# Autodesk Inventor assembly: MainAssemblie
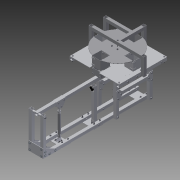
[picture p0: Inventor's stored thumbnail of the model, 180x180]
Saved by Autodesk Inventor 2013 (Build 170138000, 138)
## iProperties
Created: 2013-07-15
Part Number: MainAssemblie
Document SubType Name: Assembly
Designer: root
Mass: 9552.06 g
Surface Area: 27786.8 cm^2
Volume: 3156.7 cm^3
Density: 3.02596 g/cm^3
Author: root
## Documents named in this file (15)
- I:\FRC_Projects\Cad\Inventor_Projects\Shooter_No_Welding\MainAssemblie.iam
- I:\FRC_Projects\Cad\Inventor_Projects\Shooter_No_Welding\Base\BaseAssemblies.iam
- I:\FRC_Projects\Cad\Inventor_Projects\Shooter_No_Welding\Thrower\ThrowerAssemblie.iam
- I:\FRC_Projects\Cad\Inventor_Projects\Shooter_No_Welding\Hopper\HopperAssembly.iam
- I:\FRC_Projects\Cad\Inventor_Projects\Shooter_No_Welding\Thrower\cylinder\045_DP_D_167__F_D_166_3__2_14b.iam
- I:\FRC_Projects\Cad\Inventor_Projects\Shooter_No_Welding\Thrower\cylinder\5.ipt
- I:\FRC_Projects\Cad\Inventor_Projects\Shooter_No_Welding\Thrower\cylinder\6.ipt
- I:\FRC_Projects\Cad\Inventor_Projects\Shooter_No_Welding\contentCenter\en-US\ANSI B18.2.2(09)\ANSI B18.2.2 - 1_4 - 20(2).ipt
- I:\FRC_Projects\Cad\Inventor_Projects\Shooter_No_Welding\contentCenter\en-US\ANSI ASME B18.2.1(2)\ANSI_ASME B18.2.1 - 1_4-20 UNC - 2.25(2).ipt
- I:\FRC_Projects\Cad\Inventor_Projects\Shooter_No_Welding\contentCenter\en-US\ANSI ASME B18.2.1(2)\ANSI_ASME B18.2.1 - 1_4-20 UNC - 0.75(2).ipt
- I:\FRC_Projects\Cad\Inventor_Projects\Shooter_No_Welding\contentCenter\en-US\ASTM F436(1)\ASTM F436 - 1_4(1).ipt
- I:\FRC_Projects\Cad\Inventor_Projects\Shooter_No_Welding\Thrower\cylinder\4.ipt
- I:\FRC_Projects\Cad\Inventor_Projects\Shooter_No_Welding\contentCenter\en-US\ANSI ASME B18.2.1(2)\ANSI_ASME B18.2.1 - 1_4-20 UNC - 1.75(2).ipt
- I:\FRC_Projects\Cad\Inventor_Projects\Shooter_No_Welding\Thrower\ModdedSEN_Microswitch_V7-2B17D8-048.ipt
- I:\FRC_Projects\Cad\Inventor_Projects\Shooter_No_Welding\contentCenter\en-US\ANSI ASME B18.2.1(2)\ANSI_ASME B18.2.1 - 1_4-20 UNC - 1.5(2).ipt
## Components (43 placed, 14 different names)
1. BaseAssemblies:1 [sub-assembly] — Mate:1, Mate:2, Mate:3, Mate:4, Flush:1, Mate:7, Mate:8, Mate:9, Mate:13, Mate:18, Mate:19, Mate:23, Mate:25, Mate:27, Mate:29, Mate:30, Mate:31, Mate:32, Mate:33, Mate:34, Mate:35, Mate:36, Mate:37, Mate:38, Mate:68, Angle:1, Mate:69, Mate:70, Mate:71, Mate:72, Mate:73, Mate:74, Mate:75, Mate:76, Mate:77, Mate:82, Mate:83, Mate:84, Mate:85
2. ThrowerAssemblie:1 [sub-assembly] — Mate:1, Mate:2, Mate:11, Mate:12
3. HopperAssembly:1 [sub-assembly] — Mate:3, Mate:4, Flush:1, Mate:13, Mate:14, Mate:15, Mate:16, Mate:17, Mate:20, Mate:21, Mate:56, Mate:57, Mate:58, Mate:59, Mate:60, Mate:61, Mate:86, Mate:87, Mate:88
4. 5:1 — Mate:5, Mate:6, Flush:3, Mate:7, Mate:40, Mate:42
5. 6:1 — Mate:5, Mate:6, Flush:3, Mate:8, Mate:9, Mate:10, Mate:44, Mate:52, Mate:54, Mate:55, Flush:4
6. 045_DP_D_167__F_D_166_3__2_14b:1 [sub-assembly] — Mate:10, Mate:11, Mate:12
7. Hex Nut - Inch 1/4 - 20:1 — Mate:28, Mate:29
8. Hex Nut - Inch 1/4 - 20:2 — Mate:26, Mate:27
9. Hex Nut - Inch 1/4 - 20:3 — Mate:24, Mate:25
10. Hex Nut - Inch 1/4 - 20:4 — Mate:22, Mate:23
11. Hex Bolt - Inch 1/4-20 UNC - 2.25:1 — Mate:15, Mate:17, Mate:28
12. Hex Bolt - Inch 1/4-20 UNC - 2.25:2 — Mate:18, Mate:21, Mate:24
13. Hex Bolt - Inch 1/4-20 UNC - 2.25:3 — Mate:14, Mate:16, Mate:22
14. Hex Bolt - Inch 1/4-20 UNC - 2.25:4 — Mate:19, Mate:20, Mate:26
15. Hex Bolt - Inch 1/4-20 UNC - 0.75:1 — Mate:31, Mate:34, Mate:43, Mate:49
16. Hex Bolt - Inch 1/4-20 UNC - 0.75:2 — Mate:32, Mate:35, Mate:51, Mate:53
17. Hex Bolt - Inch 1/4-20 UNC - 0.75:3 — Mate:36
18. Hex Bolt - Inch 1/4-20 UNC - 0.75:4 — Mate:30, Mate:33, Mate:41, Mate:47
19. Hex Bolt - Inch 1/4-20 UNC - 0.75:5 — Mate:37, Mate:38, Mate:39, Mate:45
20. Hex Nut - Inch 1/4 - 20:5 — Mate:53, Mate:54
21. Hex Nut - Inch 1/4 - 20:6 — Mate:49, Mate:50
22. Hex Nut - Inch 1/4 - 20:7 — Mate:47, Mate:48
23. Hex Nut - Inch 1/4 - 20:8 — Mate:45, Mate:46
24. Circular Washer (Inch) 1/4:1 — Mate:39, Mate:40, Mate:46
25. Circular Washer (Inch) 1/4:2 — Mate:51, Mate:52
26. Circular Washer (Inch) 1/4:3 — Mate:43, Mate:44, Mate:50
27. Circular Washer (Inch) 1/4:4 — Mate:41, Mate:42, Mate:48
28. 4:1 — Mate:55, Flush:4
29. Hex Bolt - Inch 1/4-20 UNC - 1.75:1 — Mate:58, Mate:59, Mate:64
30. Hex Bolt - Inch 1/4-20 UNC - 1.75:2 — Mate:60, Mate:61, Mate:63
31. Hex Bolt - Inch 1/4-20 UNC - 1.75:3 — Mate:56, Mate:57, Mate:62
32. Hex Nut - Inch 1/4 - 20:9 — Mate:64, Mate:88
33. Hex Nut - Inch 1/4 - 20:10 — Mate:63, Mate:87
34. Hex Nut - Inch 1/4 - 20:11 — Mate:62, Mate:86
35. ModdedSEN_Microswitch_V7-2B17D8-048:1 — Mate:68, Angle:1, Mate:69
36. Hex Bolt - Inch 1/4-20 UNC - 1.5:1 — Mate:73, Mate:75, Mate:79
37. Hex Bolt - Inch 1/4-20 UNC - 1.5:2 — Mate:72, Mate:74, Mate:78
38. Hex Bolt - Inch 1/4-20 UNC - 1.5:3 — Mate:70, Mate:76, Mate:81
39. Hex Bolt - Inch 1/4-20 UNC - 1.5:4 — Mate:71, Mate:77, Mate:80
40. Hex Nut - Inch 1/4 - 20:12 — Mate:81, Mate:84
41. Hex Nut - Inch 1/4 - 20:13 — Mate:79, Mate:83
42. Hex Nut - Inch 1/4 - 20:14 — Mate:80, Mate:85
43. Hex Nut - Inch 1/4 - 20:15 — Mate:78, Mate:82
## Relationships (89: Mate 85, Flush 3, Angle 1)
- Mate:1: BaseAssemblies:1 ↔ ThrowerAssemblie:1
- Mate:2: BaseAssemblies:1 ↔ ThrowerAssemblie:1
- Mate:3: BaseAssemblies:1 ↔ HopperAssembly:1
- Mate:4: BaseAssemblies:1 ↔ HopperAssembly:1
- Flush:1: BaseAssemblies:1 ↔ HopperAssembly:1
- Mate:5 (9.525 mm): 5:1 ↔ 6:1
- Mate:6: 5:1 ↔ 6:1
- Flush:3: 5:1 ↔ 6:1
- Mate:7: BaseAssemblies:1 ↔ 5:1
- Mate:8 (184.15 mm): BaseAssemblies:1 ↔ 6:1
- Mate:9 (42.8625 mm): BaseAssemblies:1 ↔ 6:1
- Mate:10: 6:1 ↔ 045_DP_D_167__F_D_166_3__2_14b:1
- Mate:11: ThrowerAssemblie:1 ↔ 045_DP_D_167__F_D_166_3__2_14b:1
- Mate:12: ThrowerAssemblie:1 ↔ 045_DP_D_167__F_D_166_3__2_14b:1
- Mate:13: BaseAssemblies:1 ↔ HopperAssembly:1
- Mate:14: HopperAssembly:1 ↔ Hex Bolt - Inch 1/4-20 UNC - 2.25:3
- Mate:15: HopperAssembly:1 ↔ Hex Bolt - Inch 1/4-20 UNC - 2.25:1
- Mate:16: HopperAssembly:1 ↔ Hex Bolt - Inch 1/4-20 UNC - 2.25:3
- Mate:17: HopperAssembly:1 ↔ Hex Bolt - Inch 1/4-20 UNC - 2.25:1
- Mate:18: BaseAssemblies:1 ↔ Hex Bolt - Inch 1/4-20 UNC - 2.25:2
- Mate:19: BaseAssemblies:1 ↔ Hex Bolt - Inch 1/4-20 UNC - 2.25:4
- Mate:20: HopperAssembly:1 ↔ Hex Bolt - Inch 1/4-20 UNC - 2.25:4
- Mate:21: HopperAssembly:1 ↔ Hex Bolt - Inch 1/4-20 UNC - 2.25:2
- Mate:22: Hex Nut - Inch 1/4 - 20:4 ↔ Hex Bolt - Inch 1/4-20 UNC - 2.25:3
- Mate:23: BaseAssemblies:1 ↔ Hex Nut - Inch 1/4 - 20:4
- Mate:24: Hex Nut - Inch 1/4 - 20:3 ↔ Hex Bolt - Inch 1/4-20 UNC - 2.25:2
- Mate:25: BaseAssemblies:1 ↔ Hex Nut - Inch 1/4 - 20:3
- Mate:26: Hex Nut - Inch 1/4 - 20:2 ↔ Hex Bolt - Inch 1/4-20 UNC - 2.25:4
- Mate:27: BaseAssemblies:1 ↔ Hex Nut - Inch 1/4 - 20:2
- Mate:28: Hex Nut - Inch 1/4 - 20:1 ↔ Hex Bolt - Inch 1/4-20 UNC - 2.25:1
- Mate:29: BaseAssemblies:1 ↔ Hex Nut - Inch 1/4 - 20:1
- Mate:30: BaseAssemblies:1 ↔ Hex Bolt - Inch 1/4-20 UNC - 0.75:4
- Mate:31: BaseAssemblies:1 ↔ Hex Bolt - Inch 1/4-20 UNC - 0.75:1
- Mate:32: BaseAssemblies:1 ↔ Hex Bolt - Inch 1/4-20 UNC - 0.75:2
- Mate:33: BaseAssemblies:1 ↔ Hex Bolt - Inch 1/4-20 UNC - 0.75:4
- Mate:34: BaseAssemblies:1 ↔ Hex Bolt - Inch 1/4-20 UNC - 0.75:1
- Mate:35: BaseAssemblies:1 ↔ Hex Bolt - Inch 1/4-20 UNC - 0.75:2
- Mate:36: BaseAssemblies:1 ↔ Hex Bolt - Inch 1/4-20 UNC - 0.75:3
- Mate:37: BaseAssemblies:1 ↔ Hex Bolt - Inch 1/4-20 UNC - 0.75:5
- Mate:38: BaseAssemblies:1 ↔ Hex Bolt - Inch 1/4-20 UNC - 0.75:5
- Mate:39: Hex Bolt - Inch 1/4-20 UNC - 0.75:5 ↔ Circular Washer (Inch) 1/4:1
- Mate:40: 5:1 ↔ Circular Washer (Inch) 1/4:1
- Mate:41: Hex Bolt - Inch 1/4-20 UNC - 0.75:4 ↔ Circular Washer (Inch) 1/4:4
- Mate:42: 5:1 ↔ Circular Washer (Inch) 1/4:4
- Mate:43: Hex Bolt - Inch 1/4-20 UNC - 0.75:1 ↔ Circular Washer (Inch) 1/4:3
- Mate:44: 6:1 ↔ Circular Washer (Inch) 1/4:3
- Mate:45: Hex Bolt - Inch 1/4-20 UNC - 0.75:5 ↔ Hex Nut - Inch 1/4 - 20:8
- Mate:46: Hex Nut - Inch 1/4 - 20:8 ↔ Circular Washer (Inch) 1/4:1
- Mate:47: Hex Bolt - Inch 1/4-20 UNC - 0.75:4 ↔ Hex Nut - Inch 1/4 - 20:7
- Mate:48: Hex Nut - Inch 1/4 - 20:7 ↔ Circular Washer (Inch) 1/4:4
- Mate:49: Hex Bolt - Inch 1/4-20 UNC - 0.75:1 ↔ Hex Nut - Inch 1/4 - 20:6
- Mate:50: Hex Nut - Inch 1/4 - 20:6 ↔ Circular Washer (Inch) 1/4:3
- Mate:51: Hex Bolt - Inch 1/4-20 UNC - 0.75:2 ↔ Circular Washer (Inch) 1/4:2
- Mate:52: 6:1 ↔ Circular Washer (Inch) 1/4:2
- Mate:53: Hex Bolt - Inch 1/4-20 UNC - 0.75:2 ↔ Hex Nut - Inch 1/4 - 20:5
- Mate:54: 6:1 ↔ Hex Nut - Inch 1/4 - 20:5
- Mate:55: 6:1 ↔ 4:1
- Flush:4: 6:1 ↔ 4:1
- Mate:56: HopperAssembly:1 ↔ Hex Bolt - Inch 1/4-20 UNC - 1.75:3
- Mate:57: HopperAssembly:1 ↔ Hex Bolt - Inch 1/4-20 UNC - 1.75:3
- Mate:58: HopperAssembly:1 ↔ Hex Bolt - Inch 1/4-20 UNC - 1.75:1
- Mate:59: HopperAssembly:1 ↔ Hex Bolt - Inch 1/4-20 UNC - 1.75:1
- Mate:60: HopperAssembly:1 ↔ Hex Bolt - Inch 1/4-20 UNC - 1.75:2
- Mate:61: HopperAssembly:1 ↔ Hex Bolt - Inch 1/4-20 UNC - 1.75:2
- Mate:62: Hex Bolt - Inch 1/4-20 UNC - 1.75:3 ↔ Hex Nut - Inch 1/4 - 20:11
- Mate:63: Hex Bolt - Inch 1/4-20 UNC - 1.75:2 ↔ Hex Nut - Inch 1/4 - 20:10
- Mate:64: Hex Bolt - Inch 1/4-20 UNC - 1.75:1 ↔ Hex Nut - Inch 1/4 - 20:9
- Mate:68: BaseAssemblies:1 ↔ ModdedSEN_Microswitch_V7-2B17D8-048:1
- Angle:1 (-45 deg): BaseAssemblies:1 ↔ ModdedSEN_Microswitch_V7-2B17D8-048:1
- Mate:69: BaseAssemblies:1 ↔ ModdedSEN_Microswitch_V7-2B17D8-048:1
- Mate:70: BaseAssemblies:1 ↔ Hex Bolt - Inch 1/4-20 UNC - 1.5:3
- Mate:71: BaseAssemblies:1 ↔ Hex Bolt - Inch 1/4-20 UNC - 1.5:4
- Mate:72: BaseAssemblies:1 ↔ Hex Bolt - Inch 1/4-20 UNC - 1.5:2
- Mate:73: BaseAssemblies:1 ↔ Hex Bolt - Inch 1/4-20 UNC - 1.5:1
- Mate:74: BaseAssemblies:1 ↔ Hex Bolt - Inch 1/4-20 UNC - 1.5:2
- Mate:75: BaseAssemblies:1 ↔ Hex Bolt - Inch 1/4-20 UNC - 1.5:1
- Mate:76: BaseAssemblies:1 ↔ Hex Bolt - Inch 1/4-20 UNC - 1.5:3
- Mate:77: BaseAssemblies:1 ↔ Hex Bolt - Inch 1/4-20 UNC - 1.5:4
- Mate:78: Hex Bolt - Inch 1/4-20 UNC - 1.5:2 ↔ Hex Nut - Inch 1/4 - 20:15
- Mate:79: Hex Bolt - Inch 1/4-20 UNC - 1.5:1 ↔ Hex Nut - Inch 1/4 - 20:13
- Mate:80: Hex Bolt - Inch 1/4-20 UNC - 1.5:4 ↔ Hex Nut - Inch 1/4 - 20:14
- Mate:81: Hex Bolt - Inch 1/4-20 UNC - 1.5:3 ↔ Hex Nut - Inch 1/4 - 20:12
- Mate:82: BaseAssemblies:1 ↔ Hex Nut - Inch 1/4 - 20:15
- Mate:83: BaseAssemblies:1 ↔ Hex Nut - Inch 1/4 - 20:13
- Mate:84: BaseAssemblies:1 ↔ Hex Nut - Inch 1/4 - 20:12
- Mate:85: BaseAssemblies:1 ↔ Hex Nut - Inch 1/4 - 20:14
- Mate:86: HopperAssembly:1 ↔ Hex Nut - Inch 1/4 - 20:11
- Mate:87: HopperAssembly:1 ↔ Hex Nut - Inch 1/4 - 20:10
- Mate:88: HopperAssembly:1 ↔ Hex Nut - Inch 1/4 - 20:9
## Named parameters: sa_0 = -2.94472e-09, sa_1 = -4448.22, sa_2 = -1.14764e-10
note: some values were not read from the file. Shown as the stored number, unit unknown: "sa_0", "sa_1", "sa_2".
